# Autodesk Inventor assembly: CONCELEAD HINGE 170 DEG HALF OVERLAY DP45_9.5 HD1 CHDSCR
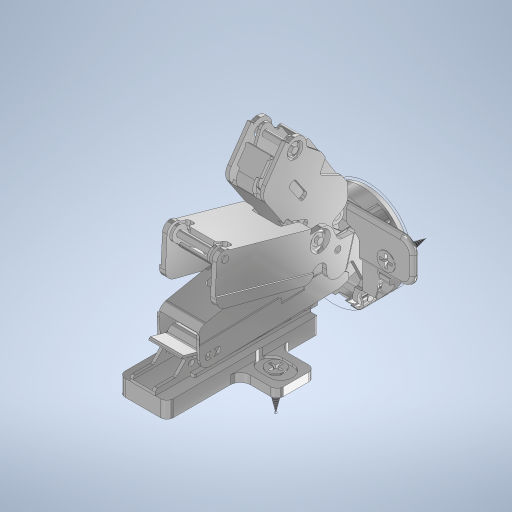
[picture p0: Inventor's stored thumbnail of the model, 512x512]
Saved by Autodesk Inventor 2024 (Build 280153000, 153)
## iProperties
Created: 2015-04-29
Part Number: CONCELEAD HINGE 170 DEG HALF OVERLAY DP45_9.5 HD1 CHDSCR
Document SubType Name: Assembly
Designer: SauliusD
Author: SauliusD
## Documents named in this file (22)
- C:\W4INV 2024 Design\LIBRARY\Hinges\CONCEALED 170 DEG HINGE HALF OVERLAY.iam
- C:\W4INV 2024 Design\LIBRARY\Hinges\Parts\170 Deg Hinge Parts\Lever 2 4 170 deg.ipt
- C:\W4INV 2024 Design\LIBRARY\Hinges\Parts\170 Deg Hinge Parts\Lever 2 3 170 deg.ipt
- C:\W4INV 2024 Design\LIBRARY\Hinges\Parts\170 Deg Hinge Parts\Lever 2 2 170 deg.ipt
- C:\W4INV 2024 Design\LIBRARY\Hinges\Parts\170 Deg Hinge Parts\Lever 2 1 170 deg.ipt
- C:\W4INV 2024 Design\LIBRARY\Hinges\Parts\170 Deg Hinge Parts\170 deg Hinge Cup.ipt
- C:\W4INV 2024 Design\LIBRARY\Hinges\Parts\170 Deg Hinge Parts\Hinge 170 Degree Half Overlay.ipt
- C:\W4INV 2024 Design\LIBRARY\Hinges\Parts\Concelead Hinge\Duomatic mounting plate .ipt
- C:\W4INV 2024 Design\LIBRARY\Hinges\Parts\170 Deg Hinge Parts\170 deg Hinge Cup\170 deg Hinge Cup DP45_9.5 HD1.ipt
- C:\W4INV 2024 Design\LIBRARY\Hinges\Parts\Concelead Hinge\Duomatic mounting plate _\Duomatic mounting plate H6 FX CHBSCR.ipt
- CONCELEAD HINGE 170 DEG HALF OVERLAY DP45_9.5 HD1 CHDSCR.iam
- CONCELEAD HINGE 170 DEG HALF OVERLAY DP45_9.5 HD1 EURSCR.iam
- CONCELEAD HINGE 170 DEG HALF OVERLAY DP45_9.5 HD8 CHDSCR.iam
- CONCELEAD HINGE 170 DEG HALF OVERLAY DP45_9.5 HD8 EURSCR.iam
- CONCELEAD HINGE 170 DEG HALF OVERLAY DP46_6 HD1 CHDSCR.iam
- CONCELEAD HINGE 170 DEG HALF OVERLAY DP46_6 HD1 EURSCR.iam
- CONCELEAD HINGE 170 DEG HALF OVERLAY DP46_6 HD10 CHDSCR.iam
- CONCELEAD HINGE 170 DEG HALF OVERLAY DP46_6 HD10 EURSCR.iam
- CONCELEAD HINGE 170 DEG HALF OVERLAY DP52_5.5 HD1 CHDSCR.iam
- CONCELEAD HINGE 170 DEG HALF OVERLAY DP52_5.5 HD1 EURSCR.iam
- CONCELEAD HINGE 170 DEG HALF OVERLAY DP52_5.5 HD10 CHDSCR.iam
- CONCELEAD HINGE 170 DEG HALF OVERLAY DP52_5.5 HD10 EURSCR.iam
## Components (7 placed, 7 different names)
1. Duomatic mounting plate H6 FX CHBSCR:1 — Flush:1, Flush:2, Flush:3, Flush:4, Flush:5, Flush:7, Angle:1
2. Hinge 170 Degree Half Overlay:1 — Flush:1, Flush:2, Mate:1, Mate:3, Flush:6, Mate:6, Mate:15, Flush:7
3. Lever 2 4 170 deg:1 — Mate:2, Mate:3, Mate:4
4. Lever 2 3 170 deg:1 — Flush:6, Mate:4, Mate:7, Mate:11
5. Lever 2 2 170 deg:1 — Mate:5, Mate:6, Mate:7, Mate:13
6. Lever 2 1 170 deg:1 — Mate:12, Mate:13, Mate:14
7. 170 deg Hinge Cup DP45_9.5 HD1:1 — Mate:9, Mate:11, Mate:14, Angle:1
## Relationships (21: Mate 13, Flush 7, Angle 1)
- Flush:1 (0.434 mm): Duomatic mounting plate H6 FX CHBSCR:1 ↔ Hinge 170 Degree Half Overlay:1
- Flush:2 (-0.549 mm): Duomatic mounting plate H6 FX CHBSCR:1 ↔ Hinge 170 Degree Half Overlay:1
- Mate:1: Hinge 170 Degree Half Overlay:1
- Flush:3: Duomatic mounting plate H6 FX CHBSCR:1
- Flush:4: Duomatic mounting plate H6 FX CHBSCR:1
- Flush:5 (3.8 mm): Duomatic mounting plate H6 FX CHBSCR:1
- Mate:2: Lever 2 4 170 deg:1
- Mate:3: Hinge 170 Degree Half Overlay:1 ↔ Lever 2 4 170 deg:1
- Flush:6: Hinge 170 Degree Half Overlay:1 ↔ Lever 2 3 170 deg:1
- Mate:4: Lever 2 4 170 deg:1 ↔ Lever 2 3 170 deg:1
- Mate:5: Lever 2 2 170 deg:1
- Mate:6: Hinge 170 Degree Half Overlay:1 ↔ Lever 2 2 170 deg:1
- Mate:7: Lever 2 3 170 deg:1 ↔ Lever 2 2 170 deg:1
- Mate:12: Lever 2 1 170 deg:1
- Mate:9: 170 deg Hinge Cup DP45_9.5 HD1:1
- Mate:11: Lever 2 3 170 deg:1 ↔ 170 deg Hinge Cup DP45_9.5 HD1:1
- Mate:13: Lever 2 2 170 deg:1 ↔ Lever 2 1 170 deg:1
- Mate:14: Lever 2 1 170 deg:1 ↔ 170 deg Hinge Cup DP45_9.5 HD1:1
- Mate:15 (18.734 mm): Hinge 170 Degree Half Overlay:1
- Flush:7 (9.851 mm): Duomatic mounting plate H6 FX CHBSCR:1 ↔ Hinge 170 Degree Half Overlay:1
- Angle:1 (270 deg): Duomatic mounting plate H6 FX CHBSCR:1 ↔ 170 deg Hinge Cup DP45_9.5 HD1:1
